# Autodesk Inventor assembly: Bielle sup v33
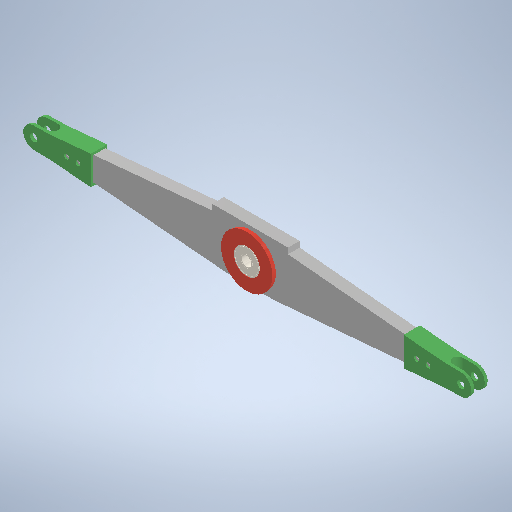
[picture p0: Inventor's stored thumbnail of the model, 512x512]
Saved by Autodesk Inventor 2025.2 (Build 292293000, 293)
## iProperties
Created: 2020-12-11
Part Number: Bielle sup v33
Document SubType Name: Assembly
Designer: genon
Title: D:/FUSION360_Export/Hub Fred j21/Project Fred/Fred/Mars Rover 2020/3Suspension/Bielle sup.f3d/Bielle sup v33.stp
Sending System: Autodesk Translation Framework v9.7.1.1290
Preprocessor: ST-DEVELOPER v18.1
## Documents named in this file (6)
- C:\Users\genon\Documents\Henallux Passerelle\Projet de conception\Cassini T-X\Inventor\Ensemble_racc_suspension.iam
- C:\Users\genon\Downloads\MarsRover2020-master\MarsRover2020-master\Mechanic\3D_CAD_Files\Individual_Parts\3Suspension\Bielle sup.f3d\Bielle sup v33\Bielle sup v33\Grande Bielle.ipt
- C:\Users\genon\Downloads\MarsRover2020-master\MarsRover2020-master\Mechanic\3D_CAD_Files\Individual_Parts\3Suspension\Bielle sup.f3d\Bielle sup v33\Bielle sup v33\Fixation rotule.ipt
- C:\Users\genon\Downloads\MarsRover2020-master\MarsRover2020-master\Mechanic\3D_CAD_Files\Individual_Parts\3Suspension\Bielle sup.f3d\Bielle sup v33\Bielle sup v33\Axe centrale V2.ipt
- C:\Users\genon\Downloads\MarsRover2020-master\MarsRover2020-master\Mechanic\3D_CAD_Files\Individual_Parts\3Suspension\Bielle sup.f3d\Bielle sup v33\Bielle sup v33\Rolling v2.ipt
- C:\Users\genon\Downloads\MarsRover2020-master\MarsRover2020-master\Mechanic\3D_CAD_Files\Individual_Parts\3Suspension\Bielle sup.f3d\Bielle sup v33\Bielle sup v33\Rolling v2 (1).ipt
## Components (7 placed, 5 different names)
1. Grande Bielle:1 — Placage:1, Placage:2, Placage:3, Placage:10, Placage:11, Placage:12, Placage:13, Placage:14, Placage:15
2. Fixation rotule:1 — Placage:13, Placage:14, Placage:15
3. Fixation rotule:2 — Placage:10, Placage:11, Placage:12
4. Axe centrale V2:1 — Placage:1, Placage:2, Placage:3, Placage:4, Placage:5, Placage:6
5. Rolling v2:1 — Placage:4, Placage:5, Placage:7
6. Axe centrale V2:3 — Placage:6, Placage:7, Placage:8, Placage:9
7. Rolling v2 (1):1 — Placage:8, Placage:9
## Relationships (15: Mate 15)
- Placage:1 [Mate]: Grande Bielle:1 ↔ Axe centrale V2:1
- Placage:2 [Mate]: Grande Bielle:1 ↔ Axe centrale V2:1
- Placage:3 [Mate]: Grande Bielle:1 ↔ Axe centrale V2:1
- Placage:4 [Mate]: Axe centrale V2:1 ↔ Rolling v2:1
- Placage:5 [Mate]: Axe centrale V2:1 ↔ Rolling v2:1
- Placage:6 [Mate]: Axe centrale V2:1 ↔ Axe centrale V2:3
- Placage:7 [Mate]: Rolling v2:1 ↔ Axe centrale V2:3
- Placage:8 [Mate]: Axe centrale V2:3 ↔ Rolling v2 (1):1
- Placage:9 [Mate]: Axe centrale V2:3 ↔ Rolling v2 (1):1
- Placage:10 [Mate]: Grande Bielle:1 ↔ Fixation rotule:2
- Placage:11 [Mate]: Grande Bielle:1 ↔ Fixation rotule:2
- Placage:12 [Mate]: Grande Bielle:1 ↔ Fixation rotule:2
- Placage:13 [Mate]: Grande Bielle:1 ↔ Fixation rotule:1
- Placage:14 [Mate]: Grande Bielle:1 ↔ Fixation rotule:1
- Placage:15 [Mate]: Grande Bielle:1 ↔ Fixation rotule:1
